# Autodesk Inventor assembly: idler_screw_join
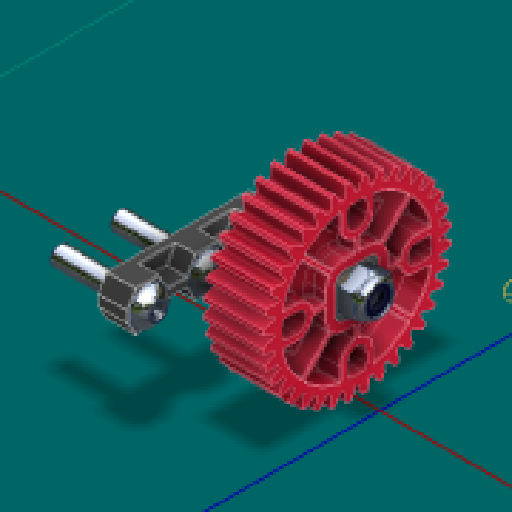
[picture p0: Inventor's stored thumbnail of the model, 512x512]
Saved by Autodesk Inventor 2025 (Build 290162000, 162)
## iProperties
Created: 2024-08-16
Part Number: idler_screw_join
Document SubType Name: Assembly
Designer: averey
Author: averey
## Documents named in this file (11)
- C:\Users\avere\vex_robotics_high_stakes\hardware\cad\ATLAS\chassis\drive_pod\gearbox\idler_screw_join.iam
- idler_screw_joint.iam
- C:\Users\avere\vex_robotics_high_stakes\hardware\cad\VEX-CAD-Inventor\Structure\Hardware\Screw Steel - Star.ipt
- C:\Users\avere\vex_robotics_high_stakes\hardware\cad\VEX-CAD-Inventor\Motion\Shaft LS\Bearing Flat Low Profile.ipt
- C:\Users\avere\vex_robotics_high_stakes\hardware\cad\VEX-CAD-Inventor\Structure\Hardware\Nut Thin Nylock.ipt
- C:\Users\avere\vex_robotics_high_stakes\hardware\cad\VEX-CAD-Inventor\Motion\Spacers\Washer Steel\SWasher .375 OD x .062500.ipt
- C:\Users\avere\vex_robotics_high_stakes\hardware\cad\VEX-CAD-Inventor\Motion\Spacers\Washer Steel.ipt
- C:\Users\avere\vex_robotics_high_stakes\hardware\cad\VEX-CAD-Inventor\Motion\Gears\HS Gear.iam
- C:\Users\avere\vex_robotics_high_stakes\hardware\cad\VEX-CAD-Inventor\Motion\Gears\HS Gear\HS 36T Gear, Circle.iam
- C:\Users\avere\vex_robotics_high_stakes\hardware\cad\VEX-CAD-Inventor\Structure\Hardware\Screw Steel - Star\SScrew Star Smooth .750.ipt
- C:\Users\avere\vex_robotics_high_stakes\hardware\cad\VEX-CAD-Inventor\Structure\Hardware\Screw Steel - Star\SScrew Star Smooth 1.500.ipt
## Components (8 placed, 6 different names)
1. Bearing Flat Low Profile:1 — Angle:1, Insert:2, Insert:6, Insert:7, Insert:8
2. Nut Thin Nylock:1 — Insert:2, Insert:3
3. SWasher .375 OD x .062500:1 — Insert:3, Insert:4
4. Nut Thin Nylock:2 — Insert:5
5. HS 36T Gear, Circle:1 [sub-assembly] — Insert:4, Insert:5
6. SScrew Star Smooth .750:2 — Insert:7
7. SScrew Star Smooth .750:3 — Insert:6
8. SScrew Star Smooth 1.500:4 — Insert:8
## Relationships (8: Insert 7, Angle 1)
- Angle:1 (0 deg): Bearing Flat Low Profile:1
- Insert:2 (1.27 mm): Bearing Flat Low Profile:1 ↔ Nut Thin Nylock:1
- Insert:3: Nut Thin Nylock:1 ↔ SWasher .375 OD x .062500:1
- Insert:4: SWasher .375 OD x .062500:1 ↔ HS 36T Gear, Circle:1
- Insert:5: Nut Thin Nylock:2 ↔ HS 36T Gear, Circle:1
- Insert:6 (1.27 mm): Bearing Flat Low Profile:1 ↔ SScrew Star Smooth .750:3
- Insert:7 (1.27 mm): Bearing Flat Low Profile:1 ↔ SScrew Star Smooth .750:2
- Insert:8 (7.9375 mm): Bearing Flat Low Profile:1 ↔ SScrew Star Smooth 1.500:4
